# Autodesk Inventor assembly: Сборка_опт_зонд_с_датчиком
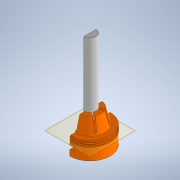
[picture p0: Inventor's stored thumbnail of the model, 180x180]
Saved by Autodesk Inventor 2021 (Build 250183000, 183)
## iProperties
Created: 2024-03-30
Part Number: Сборка_опт_зонд_с_датчиком
Document SubType Name: Assembly
Designer: Мария
Author: Мария
## Documents named in this file (7)
- D:\Documents\KiCad\8.0\projects\Learn\pressure_sensor\Разводка печатных плат_Inventor\Сборка_опт_зонд_с_датчиком.iam
- D:\Documents\Inventor\Разводка печатных плат\Оптический датчик.ipt
- D:\Documents\Inventor\Разводка печатных плат\Упор.ipt
- D:\Documents\Inventor\Разводка печатных плат\Цанга_держатель.ipt
- D:\Documents\Inventor\Разводка печатных плат\PCB\pressure_sensor_sensor2.iam
- D:\Documents\Inventor\Разводка печатных плат\PCB\pressure_sensor_logic2_.iam
- D:\Documents\Inventor\Content Center Files\R2021\ru-RU\GOST 17475-80 (2)\Винт 2.M2-6gx16 ГОСТ 17475-80.ipt
## Components (8 placed, 6 different names)
1. Оптический датчик:1 — Совмещение:6, Совмещение:11, Совмещение:12, Совмещение:18, Совмещение:19, Совмещение:20, Совмещение:23
2. Упор:1 — Совмещение:12, Совмещение:18, Совмещение:25
3. Цанга_держатель:1 — Совмещение:6, Совмещение:11, Совмещение:24, Совмещение:26, Совмещение:27, Совмещение:28, Совмещение:29, Совмещение:30, Совмещение:31
4. pressure_sensor_sensor2:1 [sub-assembly] — Совмещение:19, Совмещение:21, Совмещение:22, Совмещение:25
5. pressure_sensor_logic2_:1 [sub-assembly] — Совмещение:20, Совмещение:21, Совмещение:22, Совмещение:23, Совмещение:24
6. Винт 2 ГОСТ 17475-80 M2 x 16:1 — Совмещение:27, Совмещение:31
7. Винт 2 ГОСТ 17475-80 M2 x 16:3 — Совмещение:26, Совмещение:29
8. Винт 2 ГОСТ 17475-80 M2 x 16:2 — Совмещение:28, Совмещение:30
## Relationships (17: Mate 17)
- Совмещение:6 [Mate]: Оптический датчик:1 ↔ Цанга_держатель:1
- Совмещение:11 [Mate]: Оптический датчик:1 ↔ Цанга_держатель:1
- Совмещение:12 [Mate]: Оптический датчик:1 ↔ Упор:1
- Совмещение:18 [Mate]: Оптический датчик:1 ↔ Упор:1
- Совмещение:19 [Mate]: Оптический датчик:1 ↔ pressure_sensor_sensor2:1
- Совмещение:20 [Mate]: Оптический датчик:1 ↔ pressure_sensor_logic2_:1
- Совмещение:21 [Mate]: pressure_sensor_sensor2:1 ↔ pressure_sensor_logic2_:1
- Совмещение:22 [Mate] (4 mm): pressure_sensor_sensor2:1 ↔ pressure_sensor_logic2_:1
- Совмещение:23 [Mate]: Оптический датчик:1 ↔ pressure_sensor_logic2_:1
- Совмещение:24 [Mate]: Цанга_держатель:1 ↔ pressure_sensor_logic2_:1
- Совмещение:25 [Mate]: Упор:1 ↔ pressure_sensor_sensor2:1
- Совмещение:26 [Mate]: Цанга_держатель:1 ↔ Винт 2 ГОСТ 17475-80 M2 x 16:3
- Совмещение:27 [Mate]: Цанга_держатель:1 ↔ Винт 2 ГОСТ 17475-80 M2 x 16:1
- Совмещение:28 [Mate]: Цанга_держатель:1 ↔ Винт 2 ГОСТ 17475-80 M2 x 16:2
- Совмещение:29 [Mate]: Цанга_держатель:1 ↔ Винт 2 ГОСТ 17475-80 M2 x 16:3
- Совмещение:30 [Mate]: Цанга_держатель:1 ↔ Винт 2 ГОСТ 17475-80 M2 x 16:2
- Совмещение:31 [Mate]: Цанга_держатель:1 ↔ Винт 2 ГОСТ 17475-80 M2 x 16:1
